# Autodesk Inventor assembly: finally_we_are_done_with_stand
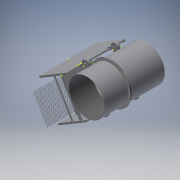
[picture p0: Inventor's stored thumbnail of the model, 180x180]
Saved by Autodesk Inventor 2019 (Build 230136000, 136)
## iProperties
Created: 2020-02-15
Part Number: finally_we_are_done_with_stand
Document SubType Name: Assembly
Designer: Admin
Author: Admin
## Documents named in this file (8)
- C:\Users\admin\Desktop\Exploration\finally_we_are_done_with_stand.iam
- C:\Users\admin\Desktop\Exploration\stand2.0.ipt
- C:\Users\admin\Desktop\Exploration\roller complete.iam
- C:\Users\admin\Desktop\Exploration\Finally_we_are_done_with_drum.ipt
- C:\Users\admin\Desktop\Exploration\grillage.ipt
- C:\Users\admin\Desktop\Exploration\DC assembly.iam
- C:\Users\admin\Desktop\Exploration\030 motor mount-2-Production.ipt
- C:\Users\admin\Desktop\Exploration\finally_we_are_done_with_stand\Design Accelerator\V-Belt transmission3.iam
## Components (10 placed, 7 different names)
1. stand2.0:1 — Rigid:1, Rigid:2, Rigid:3, Rigid:4, Rigid:5, Rigid:7, Rigid:8, Rigid:9, Angle:1
2. roller complete:1 [sub-assembly] — Rigid:1, Tangent:15
3. roller complete:2 [sub-assembly] — Rigid:2, Tangent:18
4. roller complete:3 [sub-assembly] — Rigid:3, Tangent:17
5. grillage:1 — Rigid:4, Rigid:8, Rigid:9, Angle:1
6. 030 motor mount-2-Production:1 — Rigid:5, Tangent:14, Rigid:6
7. DC assembly:1 [sub-assembly] — Tangent:14, Rigid:6
8. roller complete:4 [sub-assembly] — Rigid:7, Tangent:16
9. Finally_we_are_done_with_drum:1 — Tangent:15, Tangent:16, Tangent:17, Tangent:18
10. V-Belt transmission:1 [sub-assembly]
## Relationships (15: WeldJoint 9, Tangent 5, Angle 1)
- Rigid:1 [WeldJoint]: stand2.0:1 ↔ roller complete:1
- Rigid:2 [WeldJoint]: stand2.0:1 ↔ roller complete:2
- Rigid:3 [WeldJoint]: stand2.0:1 ↔ roller complete:3
- Rigid:4 [WeldJoint]: stand2.0:1 ↔ grillage:1
- Rigid:5 [WeldJoint]: stand2.0:1 ↔ 030 motor mount-2-Production:1
- Tangent:14: 030 motor mount-2-Production:1 ↔ DC assembly:1
- Rigid:6 [WeldJoint]: 030 motor mount-2-Production:1 ↔ DC assembly:1
- Rigid:7 [WeldJoint]: stand2.0:1 ↔ roller complete:4
- Tangent:15: roller complete:1 ↔ Finally_we_are_done_with_drum:1
- Tangent:16: roller complete:4 ↔ Finally_we_are_done_with_drum:1
- Tangent:17: roller complete:3 ↔ Finally_we_are_done_with_drum:1
- Tangent:18: roller complete:2 ↔ Finally_we_are_done_with_drum:1
- Rigid:8 [WeldJoint]: stand2.0:1 ↔ grillage:1
- Rigid:9 [WeldJoint]: stand2.0:1 ↔ grillage:1
- Angle:1 (30 deg): stand2.0:1 ↔ grillage:1
